# Autodesk Inventor assembly: Igus and Arm Bracket_MIR4
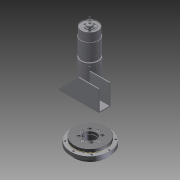
[picture p0: Inventor's stored thumbnail of the model, 180x180]
Saved by Autodesk Inventor 2015 (Build 190159000, 159)
## iProperties
Created: 2015-01-19
Part Number: Igus and Arm Bracket_MIR4
Document SubType Name: Assembly
Designer: chapale16
Author: chapale16
## Documents named in this file (4)
- \\lhssvr02\Homedirs\Robotics Club\CAD Model 2015\Igus and Arm Bracket_MIR4.iam
- \\lhssvr02\Homedirs\Robotics Club\CAD Model 2015\Game Components\The Tote Collector-Arms\Imported Components\PRT_01_30_1\PRT_01_30_1_MIR5.iam
- \\lhssvr02\Homedirs\Robotics Club\CAD Model 2015\Arm holder Bracket_MIR4.ipt
- \\lhssvr02\Homedirs\Robotics Club\CAD Model 2015\CDR prep\Tote Collector Arms\PG-71-am-0914.ipt
## Components (3 placed, 3 different names)
1. PRT_01_30_1_MIR5:1 [sub-assembly]
2. Arm holder Bracket_MIR4:1 — Mate:4, Mate:5, Angle:1, Angle:2, Mate:6
3. PG-71-am-0914:1 — Mate:4, Mate:5, Angle:1, Angle:2, Mate:6
## Relationships (5: Mate 3, Angle 2)
- Mate:4: Arm holder Bracket_MIR4:1 ↔ PG-71-am-0914:1
- Mate:5: Arm holder Bracket_MIR4:1 ↔ PG-71-am-0914:1
- Angle:1 (0 deg): Arm holder Bracket_MIR4:1 ↔ PG-71-am-0914:1
- Angle:2 (45 deg): Arm holder Bracket_MIR4:1 ↔ PG-71-am-0914:1
- Mate:6: Arm holder Bracket_MIR4:1 ↔ PG-71-am-0914:1
